# Autodesk Inventor assembly: Zespół1
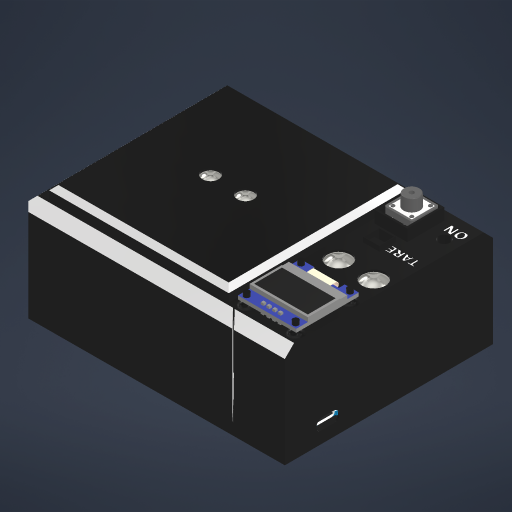
[picture p0: Inventor's stored thumbnail of the model, 512x512]
Saved by Autodesk Inventor 2024.4 (Build 284460000, 460)
## iProperties
Created: 2026-03-26
Part Number: Zespół1
Document SubType Name: Assembly
Designer: User
Author: User
## Documents named in this file (10)
- C:\Users\Duszy\Desktop\Projekty\Waga\Model\Zespół1.iam
- C:\Users\Duszy\Desktop\Projekty\Clickfy\Clickfy_V2\Clickfy_v3\loadcell_10kg_tal220B\loadcell_10kg_tal220B.ipt
- C:\Users\Duszy\Desktop\Projekty\Waga\Model\taca.ipt
- C:\Users\Duszy\Desktop\Projekty\Waga\Model\bridz.ipt
- C:\Users\Duszy\Desktop\Projekty\Waga\Model\klappa.ipt
- C:\Users\Duszy\Desktop\Projekty\Waga\Model\TP4056_Charging_Module_Type_C\TP4056_Charging_Module_Type_C\TP4056_Charging_Module_Type_C.ipt
- C:\Users\Duszy\Desktop\Projekty\Waga\Model\GUZIK.ipt
- C:\Users\Duszy\Downloads\0-9-inch-i2c-oled-128x64-display-module-1.snapshot.1\0.9 inch I2C OLED 128×64 Display Module_jhalak.ipt
- C:\Users\Duszy\Desktop\Projekty\Waga\Model\92000A328_Passivated 18-8 Stainless Steel Pan Head Phillips Screws\92000A328_Passivated 18-8 Stainless Steel Pan Head Phillips Screws\92000A328_Passivated 18-8 Stainle.ipt
- C:\Users\Duszy\Desktop\Projekty\Waga\Model\92000A220_Passivated 18-8 Stainless Steel Pan Head Phillips Screws\92000A220_Passivated 18-8 Stainless Steel Pan Head Phillips Screws\92000A220_Passivated 18-8 Stainle.ipt
## Components (11 placed, 9 different names)
1. loadcell_10kg_tal220B:1 — Obrotowe:3, Obrotowe:4, Obrotowe:5
2. taca:1 — Obrotowe:5, Obrotowe:8
3. bridz:1 — Sztywne:1, Sztywne:2
4. klappa:1 — Obrotowe:3, Obrotowe:4, Sztywne:1, Sztywne:3, Obrotowe:6, Obrotowe:7
5. TP4056_Charging_Module_Type_C:1 — Sztywne:2
6. GUZIK:1 — Obrotowe:6
7. 0.9 inch I2C OLED 128×64 Display Module_jhalak:1 — Sztywne:3
8. 92000A328_Passivated 18-8 Stainle:1 — Obrotowe:7
9. 92000A328_Passivated 18-8 Stainle:2
10. 92000A220_Passivated 18-8 Stainle:1 — Obrotowe:8
11. 92000A220_Passivated 18-8 Stainle:2
## Component patterns: (2 elements, first: 92000A328_Passivated 18-8 Stainle:1), (2 elements, first: 92000A220_Passivated 18-8 Stainle:1)
## Relationships (9: RevoluteJoint 6, WeldJoint 3)
- Obrotowe:3 [RevoluteJoint]: loadcell_10kg_tal220B:1 ↔ klappa:1
- Obrotowe:4 [RevoluteJoint]: loadcell_10kg_tal220B:1 ↔ klappa:1
- Obrotowe:5 [RevoluteJoint]: loadcell_10kg_tal220B:1 ↔ taca:1
- Sztywne:1 [WeldJoint] (12.7 mm): bridz:1 ↔ klappa:1
- Sztywne:2 [WeldJoint] (0.4 mm): bridz:1 ↔ TP4056_Charging_Module_Type_C:1
- Sztywne:3 [WeldJoint] (-3 mm): klappa:1 ↔ 0.9 inch I2C OLED 128×64 Display Module_jhalak:1
- Obrotowe:6 [RevoluteJoint] (-2 mm): klappa:1 ↔ GUZIK:1
- Obrotowe:7 [RevoluteJoint] (-21 mm): klappa:1 ↔ 92000A328_Passivated 18-8 Stainle:1
- Obrotowe:8 [RevoluteJoint] (-10 mm): taca:1 ↔ 92000A220_Passivated 18-8 Stainle:1
